# Autodesk Inventor assembly: Сборка полная
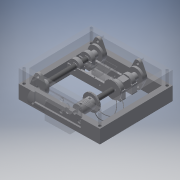
[picture p0: Inventor's stored thumbnail of the model, 180x180]
Saved by Autodesk Inventor 2017 (Build 210142000, 142)
## iProperties
Part Number: Сборка полная
Material: Типовые
Document SubType Name: Assembly
Designer: Daemon
Author: Daemon
## Documents named in this file (13)
- C:\Users\Daemon\Documents\БУ двигателем\Сборка полная.iam
- C:\Users\Daemon\Documents\БУ двигателем\Корпус низ.ipt
- C:\Users\Daemon\Documents\БУ двигателем\KFL08.ipt
- C:\Users\Daemon\Documents\БУ двигателем\Муфта4х5_ЗЕРКАЛО.ipt
- C:\Users\Daemon\Documents\БУ двигателем\Направляющая.ipt
- C:\Users\Daemon\Documents\БУ двигателем\KFL08_ЗЕРКАЛО1.ipt
- C:\Users\Daemon\Documents\БУ двигателем\KFL08_ЗЕРКАЛО2.ipt
- C:\Users\Daemon\Documents\БУ двигателем\Сборка водила.iam
- C:\Users\Daemon\Documents\БУ двигателем\Нагаечник.ipt
- C:\Users\Daemon\Documents\БУ двигателем\Крепление.ipt
- C:\Users\Daemon\Documents\БУ двигателем\Петля.ipt
- C:\Users\Daemon\Documents\БУ двигателем\Мотор.ipt
- C:\Users\Daemon\Documents\БУ двигателем\Корпус низ_ЗЕРКАЛО.ipt
## Components (15 placed, 12 different names)
1. Корпус низ:1 — С поворотом:4, С поворотом:5, С поворотом:6, С поворотом:8, С поворотом:9, Совмещение:5, Цилиндрический:13, Цилиндрический:14, Цилиндрический:15, Цилиндрический:16, Совмещение:6
2. Муфта4х5_ЗЕРКАЛО:1 — Цилиндрический:12, Совмещение:5, Жесткий:2, С поворотом:10
3. KFL08:1 — С поворотом:4, Жесткий:1
4. KFL08_ЗЕРКАЛО1:1 — С поворотом:5, Цилиндрический:1
5. Направляющая:1 — Жесткий:1, Цилиндрический:1, Цилиндрический:4
6. KFL08_ЗЕРКАЛО2:1 — С поворотом:6, Цилиндрический:2
7. Направляющая:2 — Цилиндрический:2, Цилиндрический:3, Цилиндрический:5, Цилиндрический:6, Цилиндрический:7, Жесткий:2
8. Сборка водила:1 [sub-assembly] — Цилиндрический:3, Цилиндрический:4, Совмещение:1, Совмещение:2
9. Нагаечник:1 — Цилиндрический:5, Совмещение:1
10. Крепление:1 — Цилиндрический:6, Цилиндрический:8, Совмещение:3, Цилиндрический:10, Совмещение:4, С поворотом:10
11. Крепление:2 — Цилиндрический:7, Совмещение:2, Цилиндрический:9, Цилиндрический:11
12. Петля:1 — Цилиндрический:8, Цилиндрический:9, Совмещение:3
13. Петля:2 — Цилиндрический:10, Цилиндрический:11, Совмещение:4
14. Мотор:1 — С поворотом:8, С поворотом:9, Цилиндрический:12
15. Корпус низ_ЗЕРКАЛО:1 — Цилиндрический:13, Цилиндрический:14, Цилиндрический:15, Цилиндрический:16, Совмещение:6
## Relationships (30: CylindricalJoint 16, RevoluteJoint 6, Mate 6, WeldJoint 2)
- С поворотом:4 [RevoluteJoint]: Корпус низ:1 ↔ KFL08:1
- С поворотом:5 [RevoluteJoint]: Корпус низ:1 ↔ KFL08_ЗЕРКАЛО1:1
- Жесткий:1 [WeldJoint]: KFL08:1 ↔ Направляющая:1
- Цилиндрический:1 [CylindricalJoint]: KFL08_ЗЕРКАЛО1:1 ↔ Направляющая:1
- С поворотом:6 [RevoluteJoint]: Корпус низ:1 ↔ KFL08_ЗЕРКАЛО2:1
- Цилиндрический:2 [CylindricalJoint]: KFL08_ЗЕРКАЛО2:1 ↔ Направляющая:2
- Цилиндрический:3 [CylindricalJoint]: Направляющая:2 ↔ Сборка водила:1
- Цилиндрический:4 [CylindricalJoint]: Направляющая:1 ↔ Сборка водила:1
- Цилиндрический:5 [CylindricalJoint]: Направляющая:2 ↔ Нагаечник:1
- Совмещение:1 [Mate]: Сборка водила:1 ↔ Нагаечник:1
- Цилиндрический:6 [CylindricalJoint]: Направляющая:2 ↔ Крепление:1
- Цилиндрический:7 [CylindricalJoint]: Направляющая:2 ↔ Крепление:2
- Совмещение:2 [Mate]: Сборка водила:1 ↔ Крепление:2
- Цилиндрический:8 [CylindricalJoint]: Крепление:1 ↔ Петля:1
- Цилиндрический:9 [CylindricalJoint]: Крепление:2 ↔ Петля:1
- Совмещение:3 [Mate]: Крепление:1 ↔ Петля:1
- Цилиндрический:10 [CylindricalJoint]: Крепление:1 ↔ Петля:2
- Цилиндрический:11 [CylindricalJoint]: Крепление:2 ↔ Петля:2
- Совмещение:4 [Mate]: Крепление:1 ↔ Петля:2
- С поворотом:8 [RevoluteJoint]: Корпус низ:1 ↔ Мотор:1
- С поворотом:9 [RevoluteJoint]: Корпус низ:1 ↔ Мотор:1
- Цилиндрический:12 [CylindricalJoint]: Муфта4х5_ЗЕРКАЛО:1 ↔ Мотор:1
- Совмещение:5 [Mate]: Корпус низ:1 ↔ Муфта4х5_ЗЕРКАЛО:1
- Жесткий:2 [WeldJoint]: Муфта4х5_ЗЕРКАЛО:1 ↔ Направляющая:2
- С поворотом:10 [RevoluteJoint]: Муфта4х5_ЗЕРКАЛО:1 ↔ Крепление:1
- Цилиндрический:13 [CylindricalJoint]: Корпус низ:1 ↔ Корпус низ_ЗЕРКАЛО:1
- Цилиндрический:14 [CylindricalJoint]: Корпус низ:1 ↔ Корпус низ_ЗЕРКАЛО:1
- Цилиндрический:15 [CylindricalJoint]: Корпус низ:1 ↔ Корпус низ_ЗЕРКАЛО:1
- Цилиндрический:16 [CylindricalJoint]: Корпус низ:1 ↔ Корпус низ_ЗЕРКАЛО:1
- Совмещение:6 [Mate]: Корпус низ:1 ↔ Корпус низ_ЗЕРКАЛО:1
